# Autodesk Inventor assembly: M2-ashi-unit
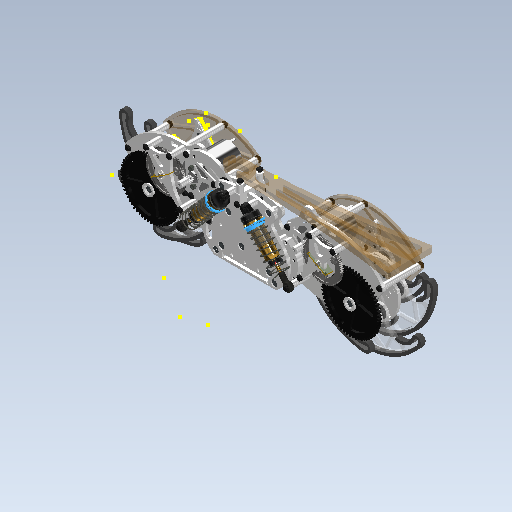
[picture p0: Inventor's stored thumbnail of the model, 512x512]
Saved by Autodesk Inventor 2020.4 (Build 244396000, 396)
## iProperties
Created: 2021-02-23
Part Number: M2-ashi-unit
Document SubType Name: Assembly
Designer: AA19065
Mass: 833.018 g
Surface Area: 3123.14 cm^2
Volume: 276.701 cm^3
Density: 3.01054 g/cm^3
Author: AA19065
## Documents named in this file (24)
- C:\Users\happy\OneDrive\ドキュメント\賢一ファイル\SRDC\試作10-2\アセンブリ\M2-ashi-unit.iam
- C:\Users\happy\OneDrive\ドキュメント\賢一ファイル\SRDC\試作10-2\アセンブリ\M2-前足.iam
- C:\Users\happy\OneDrive\ドキュメント\賢一ファイル\SRDC\試作10-2\アセンブリ\M2-M-前足.iam
- C:\Users\happy\OneDrive\ドキュメント\賢一ファイル\SRDC\試作10-2\フレーム\M2-脚中間フレーム内v2.ipt
- C:\Users\happy\OneDrive\ドキュメント\賢一ファイル\SRDC\試作10-2\フレーム\M2-脚中間フレーム外v2.ipt
- C:\Users\happy\OneDrive\ドキュメント\賢一ファイル\SRDC\試作10-2\スペーサ\M2-5mm.ipt
- C:\Users\happy\OneDrive\ドキュメント\賢一ファイル\SRDC\試作10-2\ねじ\M2-m3皿ネジ5 (1).ipt
- C:\Users\happy\OneDrive\ドキュメント\賢一ファイル\SRDC\試作10-2\フレーム\M2-アンノーン後.ipt
- C:\Users\happy\OneDrive\ドキュメント\賢一ファイル\SRDC\試作10-2\フレーム\M2-アンノーン前.ipt
- C:\Users\happy\OneDrive\ドキュメント\賢一ファイル\SRDC\試作10-2\スペーサ\M2-12mm.ipt
- C:\Users\happy\OneDrive\ドキュメント\賢一ファイル\SRDC\試作10-2\ねじ\M2-M3ボタンボルト8.ipt
- C:\Users\happy\OneDrive\ドキュメント\賢一ファイル\SRDC\試作10-2\フレーム\M2-heiko-ue.ipt
- C:\Users\happy\OneDrive\ドキュメント\賢一ファイル\SRDC\試作10-2\フレーム\M2-hieko-sita.ipt
- C:\Users\happy\OneDrive\ドキュメント\賢一ファイル\SRDC\試作10-2\軸受け\M2-オイレスw3f6-8a.ipt
- C:\Users\happy\OneDrive\ドキュメント\賢一ファイル\SRDC\試作10-2\軸受け\M2-オイレスw1.5f6-8n.ipt
- C:\Users\happy\OneDrive\ドキュメント\賢一ファイル\SRDC\試作10-2\ねじ\M2-ワッシャ3-8  0.5.ipt
- C:\Users\happy\OneDrive\ドキュメント\賢一ファイル\SRDC\試作10-2\スペーサ\M2-18mm.ipt
- C:\Users\happy\OneDrive\ドキュメント\賢一ファイル\SRDC\試作10-2\アセンブリ\M2-タミヤダンパー1.iam
- C:\Users\happy\OneDrive\ドキュメント\賢一ファイル\SRDC\試作10-2\スペーサ\M2-8mm.ipt
- C:\Users\happy\OneDrive\ドキュメント\賢一ファイル\SRDC\試作10-2\ねじ\M2-M3ボタンボルト20.ipt
- C:\Users\happy\OneDrive\ドキュメント\賢一ファイル\SRDC\試作10-2\ウィング\M2-ウィング土台.ipt
- C:\Users\happy\OneDrive\ドキュメント\賢一ファイル\SRDC\試作10-2\ウィング\M2-wing.ipt
- C:\Users\happy\OneDrive\ドキュメント\賢一ファイル\SRDC\試作10-2\ウィング\M2-ウィングおさえ.ipt
- C:\Users\happy\OneDrive\ドキュメント\賢一ファイル\SRDC\試作10-2\ねじ\M2-M3ボタンボルト12.ipt
## Components (69 placed, 23 different names)
1. M2-前足:1 [sub-assembly] — 挿入:48, 挿入:50, 挿入:54, 挿入:62, 挿入:70
2. M2-M-前足:1 [sub-assembly] — 挿入:33, 挿入:61, 挿入:69
3. M2-脚中間フレーム内v2:1 — 挿入:1, 挿入:4, 挿入:2, 挿入:3, 挿入:7, 挿入:8, 挿入:9, 挿入:11, 挿入:12, 挿入:13, 挿入:14, 挿入:10, 挿入:15, 挿入:16, 挿入:26, 挿入:24, 挿入:25, 挿入:23, 挿入:22, 挿入:21, メイト:5, メイト:6, 挿入:63, 挿入:64, メイト:9
4. M2-脚中間フレーム外v2:1 — 挿入:5, 挿入:6, 挿入:20, 挿入:19, 挿入:18, 挿入:17, メイト:2, メイト:8, メイト:7
5. M2-5mm:1 — 挿入:5, 挿入:1, メイト:3
6. M2-5mm:2 — 挿入:6, 挿入:4
7. M2-5mm:3 — 挿入:2
8. M2-5mm:4 — 挿入:3
9. M2-m3皿ネジ5 (1):1 — 挿入:7
10. M2-m3皿ネジ5 (1):2 — 挿入:8
11. M2-m3皿ネジ5 (1):3 — 挿入:9
12. M2-m3皿ネジ5 (1):4 — 挿入:11
13. M2-m3皿ネジ5 (1):5 — 挿入:12
14. M2-m3皿ネジ5 (1):6 — 挿入:13
15. M2-m3皿ネジ5 (1):7 — 挿入:14
16. M2-m3皿ネジ5 (1):8 — 挿入:10
17. M2-m3皿ネジ5 (1):9 — 挿入:15
18. M2-m3皿ネジ5 (1):10 — 挿入:16
19. M2-m3皿ネジ5 (1):11 — 挿入:20
20. M2-m3皿ネジ5 (1):12 — 挿入:19
21. M2-m3皿ネジ5 (1):13 — 挿入:18
22. M2-m3皿ネジ5 (1):14 — 挿入:17
23. M2-アンノーン後:1 — 挿入:29, 挿入:30, 挿入:39, 挿入:38, 挿入:37
24. M2-アンノーン前:1 — 挿入:32, 挿入:31, 挿入:36, 挿入:34, 挿入:35
25. M2-12mm:1 — 挿入:32, 挿入:26
26. M2-12mm:2 — 挿入:31, 挿入:24
27. M2-12mm:3 — 挿入:25, メイト:1
28. M2-12mm:4 — 挿入:29, 挿入:23
29. M2-12mm:5 — 挿入:33, 挿入:22
30. M2-12mm:6 — 挿入:30, 挿入:21
31. M2-M3ボタンボルト8:1 — 挿入:39
32. M2-M3ボタンボルト8:2 — 挿入:38
33. M2-M3ボタンボルト8:3 — 挿入:36
34. M2-M3ボタンボルト8:4 — 挿入:37
35. M2-M3ボタンボルト8:5 — 挿入:34
36. M2-M3ボタンボルト8:6 — 挿入:35
37. M2-heiko-ue:1 — メイト:2, 挿入:49, 挿入:46
38. M2-hieko-sita:1 — 挿入:41, 挿入:51
39. M2-オイレスw3f6-8a:1 — メイト:1, 挿入:41
40. M2-オイレスw3f6-8a:2 — メイト:3, 挿入:49
41. M2-5mm:5 — 挿入:46, 挿入:47, 挿入:53
42. M2-オイレスw3f6-8a:3 — 挿入:48, 挿入:47
43. M2-オイレスw1.5f6-8n:1 — 挿入:51, 挿入:50
44. M2-M3ボタンボルト8:7 — 挿入:52
45. M2-ワッシャ3-8  0.5:1 — 挿入:53, 挿入:52
46. M2-18mm:1 — 挿入:54, 挿入:71, 挿入:58
47. M2-M3ボタンボルト8:8 — 挿入:55
48. M2-ワッシャ3-8  0.5:2 — 挿入:71, 挿入:55
49. M2-M3ボタンボルト8:9 — 挿入:56
50. M2-ワッシャ3-8  0.5:3 — 挿入:58, 挿入:56
51. M2-タミヤダンパー1:1 [sub-assembly] — 挿入:61, メイト:5, 挿入:66, 挿入:68
52. M2-タミヤダンパー1:2 [sub-assembly] — 挿入:62, メイト:6, 挿入:65, 挿入:67
53. M2-8mm:1 — 挿入:63
54. M2-8mm:2 — 挿入:64
55. M2-M3ボタンボルト20:1 — 挿入:65
56. M2-M3ボタンボルト20:2 — 挿入:66
57. M2-M3ボタンボルト8:10 — 挿入:68
58. M2-M3ボタンボルト8:11 — 挿入:67
59. M2-M3ボタンボルト8:12 — 挿入:69
60. M2-M3ボタンボルト8:13 — 挿入:70
61. M2-ウィング土台:1 — メイト:9, メイト:8, メイト:7, 挿入:72, 挿入:73, 挿入:79, 挿入:80
62. M2-8mm:3 — 挿入:72, 挿入:74, 挿入:75
63. M2-8mm:4 — 挿入:73, 挿入:76
64. M2-wing:1 — 挿入:74
65. M2-ウィングおさえ:1 — 挿入:76, 挿入:75, 挿入:78, 挿入:77
66. M2-M3ボタンボルト12:1 — 挿入:79
67. M2-M3ボタンボルト12:2 — 挿入:78
68. M2-M3ボタンボルト12:3 — 挿入:77
69. M2-M3ボタンボルト12:4 — 挿入:80
## Relationships (78: Insert 70, Mate 8)
- 挿入:5 [Insert]: M2-脚中間フレーム外v2:1 ↔ M2-5mm:1
- 挿入:1 [Insert]: M2-脚中間フレーム内v2:1 ↔ M2-5mm:1
- 挿入:6 [Insert]: M2-脚中間フレーム外v2:1 ↔ M2-5mm:2
- 挿入:4 [Insert]: M2-脚中間フレーム内v2:1 ↔ M2-5mm:2
- 挿入:2 [Insert]: M2-脚中間フレーム内v2:1 ↔ M2-5mm:3
- 挿入:3 [Insert]: M2-脚中間フレーム内v2:1 ↔ M2-5mm:4
- 挿入:7 [Insert]: M2-脚中間フレーム内v2:1 ↔ M2-m3皿ネジ5 (1):1
- 挿入:8 [Insert]: M2-脚中間フレーム内v2:1 ↔ M2-m3皿ネジ5 (1):2
- 挿入:9 [Insert]: M2-脚中間フレーム内v2:1 ↔ M2-m3皿ネジ5 (1):3
- 挿入:11 [Insert]: M2-脚中間フレーム内v2:1 ↔ M2-m3皿ネジ5 (1):4
- 挿入:12 [Insert]: M2-脚中間フレーム内v2:1 ↔ M2-m3皿ネジ5 (1):5
- 挿入:13 [Insert]: M2-脚中間フレーム内v2:1 ↔ M2-m3皿ネジ5 (1):6
- 挿入:14 [Insert]: M2-脚中間フレーム内v2:1 ↔ M2-m3皿ネジ5 (1):7
- 挿入:10 [Insert]: M2-脚中間フレーム内v2:1 ↔ M2-m3皿ネジ5 (1):8
- 挿入:15 [Insert]: M2-脚中間フレーム内v2:1 ↔ M2-m3皿ネジ5 (1):9
- 挿入:16 [Insert]: M2-脚中間フレーム内v2:1 ↔ M2-m3皿ネジ5 (1):10
- 挿入:20 [Insert]: M2-脚中間フレーム外v2:1 ↔ M2-m3皿ネジ5 (1):11
- 挿入:19 [Insert]: M2-脚中間フレーム外v2:1 ↔ M2-m3皿ネジ5 (1):12
- 挿入:18 [Insert]: M2-脚中間フレーム外v2:1 ↔ M2-m3皿ネジ5 (1):13
- 挿入:17 [Insert]: M2-脚中間フレーム外v2:1 ↔ M2-m3皿ネジ5 (1):14
- 挿入:32 [Insert]: M2-アンノーン前:1 ↔ M2-12mm:1
- 挿入:26 [Insert]: M2-脚中間フレーム内v2:1 ↔ M2-12mm:1
- 挿入:31 [Insert]: M2-アンノーン前:1 ↔ M2-12mm:2
- 挿入:24 [Insert]: M2-脚中間フレーム内v2:1 ↔ M2-12mm:2
- 挿入:25 [Insert]: M2-脚中間フレーム内v2:1 ↔ M2-12mm:3
- 挿入:29 [Insert]: M2-アンノーン後:1 ↔ M2-12mm:4
- 挿入:23 [Insert]: M2-脚中間フレーム内v2:1 ↔ M2-12mm:4
- 挿入:33 [Insert]: M2-M-前足:1 ↔ M2-12mm:5
- 挿入:22 [Insert]: M2-脚中間フレーム内v2:1 ↔ M2-12mm:5
- 挿入:30 [Insert]: M2-アンノーン後:1 ↔ M2-12mm:6
- 挿入:21 [Insert]: M2-脚中間フレーム内v2:1 ↔ M2-12mm:6
- 挿入:39 [Insert]: M2-アンノーン後:1 ↔ M2-M3ボタンボルト8:1
- 挿入:38 [Insert]: M2-アンノーン後:1 ↔ M2-M3ボタンボルト8:2
- 挿入:36 [Insert]: M2-アンノーン前:1 ↔ M2-M3ボタンボルト8:3
- 挿入:37 [Insert]: M2-アンノーン後:1 ↔ M2-M3ボタンボルト8:4
- 挿入:34 [Insert]: M2-アンノーン前:1 ↔ M2-M3ボタンボルト8:5
- 挿入:35 [Insert]: M2-アンノーン前:1 ↔ M2-M3ボタンボルト8:6
- メイト:2 [Mate]: M2-脚中間フレーム外v2:1 ↔ M2-heiko-ue:1
- メイト:1 [Mate]: M2-12mm:3 ↔ M2-オイレスw3f6-8a:1
- 挿入:41 [Insert]: M2-hieko-sita:1 ↔ M2-オイレスw3f6-8a:1
- メイト:3 [Mate]: M2-5mm:1 ↔ M2-オイレスw3f6-8a:2
- 挿入:49 [Insert]: M2-heiko-ue:1 ↔ M2-オイレスw3f6-8a:2
- 挿入:46 [Insert]: M2-heiko-ue:1 ↔ M2-5mm:5
- 挿入:48 [Insert]: M2-前足:1 ↔ M2-オイレスw3f6-8a:3
- 挿入:47 [Insert] (1 mm): M2-5mm:5 ↔ M2-オイレスw3f6-8a:3
- 挿入:51 [Insert]: M2-hieko-sita:1 ↔ M2-オイレスw1.5f6-8n:1
- 挿入:50 [Insert]: M2-前足:1 ↔ M2-オイレスw1.5f6-8n:1
- 挿入:53 [Insert]: M2-5mm:5 ↔ M2-ワッシャ3-8  0.5:1
- 挿入:52 [Insert]: M2-M3ボタンボルト8:7 ↔ M2-ワッシャ3-8  0.5:1
- 挿入:54 [Insert] (-3.5 mm): M2-前足:1 ↔ M2-18mm:1
- 挿入:71 [Insert]: M2-18mm:1 ↔ M2-ワッシャ3-8  0.5:2
- 挿入:55 [Insert]: M2-M3ボタンボルト8:8 ↔ M2-ワッシャ3-8  0.5:2
- 挿入:58 [Insert]: M2-18mm:1 ↔ M2-ワッシャ3-8  0.5:3
- 挿入:56 [Insert]: M2-M3ボタンボルト8:9 ↔ M2-ワッシャ3-8  0.5:3
- 挿入:61 [Insert]: M2-M-前足:1 ↔ M2-タミヤダンパー1:1
- メイト:5 [Mate]: M2-脚中間フレーム内v2:1 ↔ M2-タミヤダンパー1:1
- 挿入:62 [Insert]: M2-前足:1 ↔ M2-タミヤダンパー1:2
- メイト:6 [Mate]: M2-脚中間フレーム内v2:1 ↔ M2-タミヤダンパー1:2
- 挿入:63 [Insert]: M2-脚中間フレーム内v2:1 ↔ M2-8mm:1
- 挿入:64 [Insert]: M2-脚中間フレーム内v2:1 ↔ M2-8mm:2
- 挿入:65 [Insert]: M2-タミヤダンパー1:2 ↔ M2-M3ボタンボルト20:1
- 挿入:66 [Insert]: M2-タミヤダンパー1:1 ↔ M2-M3ボタンボルト20:2
- 挿入:68 [Insert]: M2-タミヤダンパー1:1 ↔ M2-M3ボタンボルト8:10
- 挿入:67 [Insert]: M2-タミヤダンパー1:2 ↔ M2-M3ボタンボルト8:11
- 挿入:69 [Insert]: M2-M-前足:1 ↔ M2-M3ボタンボルト8:12
- 挿入:70 [Insert]: M2-前足:1 ↔ M2-M3ボタンボルト8:13
- メイト:9 [Mate]: M2-脚中間フレーム内v2:1 ↔ M2-ウィング土台:1
- メイト:8 [Mate]: M2-脚中間フレーム外v2:1 ↔ M2-ウィング土台:1
- メイト:7 [Mate]: M2-脚中間フレーム外v2:1 ↔ M2-ウィング土台:1
- 挿入:72 [Insert]: M2-ウィング土台:1 ↔ M2-8mm:3
- 挿入:73 [Insert]: M2-ウィング土台:1 ↔ M2-8mm:4
- 挿入:74 [Insert]: M2-8mm:3 ↔ M2-wing:1
- 挿入:76 [Insert]: M2-8mm:4 ↔ M2-ウィングおさえ:1
- 挿入:75 [Insert]: M2-8mm:3 ↔ M2-ウィングおさえ:1
- 挿入:79 [Insert]: M2-ウィング土台:1 ↔ M2-M3ボタンボルト12:1
- 挿入:78 [Insert]: M2-ウィングおさえ:1 ↔ M2-M3ボタンボルト12:2
- 挿入:77 [Insert]: M2-ウィングおさえ:1 ↔ M2-M3ボタンボルト12:3
- 挿入:80 [Insert]: M2-ウィング土台:1 ↔ M2-M3ボタンボルト12:4
